# Autodesk Inventor assembly: AM14U Long Half
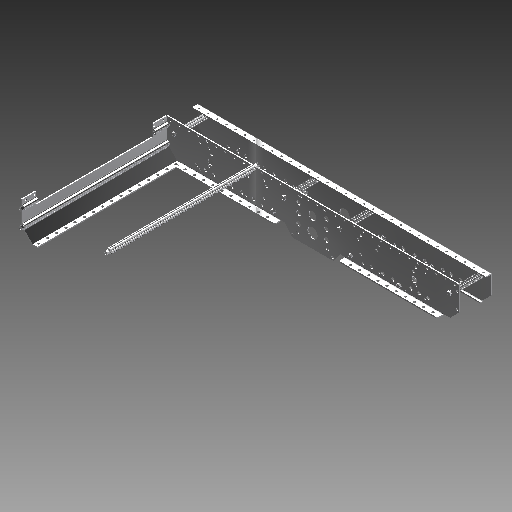
[picture p0: Inventor's stored thumbnail of the model, 512x512]
Saved by Autodesk Inventor 2017 (Build 210142000, 142)
## iProperties
Created: 2014-01-08
Part Number: AM14U Long Half
Document SubType Name: Assembly
Designer: 300593
Mass: 2039.11 g
Surface Area: 5346.56 cm^2
Volume: 755.227 cm^3
Density: 2.7 g/cm^3
Author: 300593
## Documents named in this file (7)
- \\Mac\Home\Desktop\bunnybots 2016\15102898-16-Bunnybot-CAD\Bunnybot-To_be_renamed\15102898-16-A-0000\15102898-16-A-0100\AM14U Long Half.iam
- \\Mac\Home\Desktop\bunnybots 2016\15102898-16-Bunnybot-CAD\Bunnybot-To_be_renamed\15102898-16-A-0000\15102898-16-A-0100\Churro 3375 and Screws.iam
- \\Mac\Home\Desktop\bunnybots 2016\15102898-16-Bunnybot-CAD\Bunnybot-To_be_renamed\15102898-16-A-0000\15102898-16-A-0100\Outside Plate - Master.ipt
- \\Mac\Home\Desktop\bunnybots 2016\15102898-16-Bunnybot-CAD\Bunnybot-To_be_renamed\15102898-16-A-0000\15102898-16-A-0100\Cross Brace Extrusion 15-75.ipt
- \\Mac\Home\Desktop\bunnybots 2016\15102898-16-Bunnybot-CAD\Bunnybot-To_be_renamed\15102898-16-A-0000\15102898-16-A-0100\Churro cross link and Screws.iam
- \\Mac\Home\Desktop\bunnybots 2016\15102898-16-Bunnybot-CAD\Bunnybot-To_be_renamed\15102898-16-A-0000\15102898-16-A-0100\FHTS 0.25-20-0.75_FHTS 0.25-20-G-0.75-C.ipt
- \\Mac\Home\Desktop\bunnybots 2016\15102898-16-Bunnybot-CAD\Bunnybot-To_be_renamed\15102898-16-A-0000\15102898-16-A-0100\Inside Plate - Master.ipt
## Components (16 placed, 6 different names)
1. Churro 3375 and Screws:1 [sub-assembly]
2. Outside Plate - Master:1
3. Cross Brace Extrusion 15-75:1
4. Churro 3375 and Screws:2 [sub-assembly]
5. Churro 3375 and Screws:3 [sub-assembly]
6. Churro 3375 and Screws:4 [sub-assembly]
7. Churro 3375 and Screws:5 [sub-assembly]
8. Churro 3375 and Screws:6 [sub-assembly]
9. Churro cross link and Screws:1 [sub-assembly] — Mate:1
10. FHTS 0.25-20-0.75_FHTS 0.25-20-G-0.75-C:1
11. Churro 3375 and Screws:7 [sub-assembly]
12. FHTS 0.25-20-0.75_FHTS 0.25-20-G-0.75-C:2
13. Churro 3375 and Screws:8 [sub-assembly]
14. FHTS 0.25-20-0.75_FHTS 0.25-20-G-0.75-C:3
15. FHTS 0.25-20-0.75_FHTS 0.25-20-G-0.75-C:4
16. Inside Plate - Master:1 — Mate:1
## Relationships (1: Mate 1)
- Mate:1: Churro cross link and Screws:1 ↔ Inside Plate - Master:1
